# Autodesk Inventor assembly: Gearbox - 54 to 1
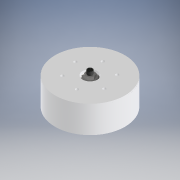
[picture p0: Inventor's stored thumbnail of the model, 180x180]
Saved by Autodesk Inventor 2017 SP1 (Build 210196100, 196)
## iProperties
Created: 2017-09-22
Part Number: Gearbox - 54 to 1
Document SubType Name: Assembly
Designer: Zach
Author: Zach
## Documents named in this file (10)
- C:\Users\Zach\Documents\GitHub\tr1\lib\Gearbox 128;1\Gearbox 128;1.iam
- C:\Users\Zach\Documents\GitHub\tr1\lib\Gearbox 128;1\Base.ipt
- C:\Users\Zach\Documents\GitHub\tr1\lib\22x8x8mm Bearing.ipt
- C:\Users\Zach\Documents\GitHub\tr1\lib\Gearbox 128;1\3mm Brass Rod.ipt
- C:\Users\Zach\Documents\Inventor\Content Center Files\R2017\en-US\ISO 4018\ISO 4018 - M8 x 50.ipt
- C:\Users\Zach\Documents\GitHub\tr1\lib\CNS 3129 - M 8 x 1.25.ipt
- C:\Users\Zach\Documents\GitHub\tr1\lib\Gearbox 128;1\Washer.ipt
- C:\Users\Zach\Documents\GitHub\tr1\lib\Gearbox 128;1\GearSet 1.iam
- C:\Users\Zach\Documents\GitHub\tr1\lib\Gearbox 128;1\Cover.ipt
- C:\Users\Zach\Documents\GitHub\tr1\lib\Gearbox 128;1\Design Accelerator\Spur Gear11.ipt
## Components (34 placed, 9 different names)
1. Base:1 — Mate:1, Flush:1, Mate:4, Flush:2, Mate:5, Flush:3, Mate:6, Flush:4, Mate:7, Flush:5, Mate:8, Flush:6, Mate:9, Flush:7
2. Cover — Mate:155, Flush:14, Mate:157, Rotation:11
3. 22x8x8mm Bearing:1 — Mate:1, Flush:1, Mate:2, Mate:63, Mate:143
4. ISO 4018 M8 x 50:1 — Mate:2, Mate:63, Mate:105, Mate:142, Rotation:7, Mate:155, Mate:156
5. 3mm Brass Rod:1 — Mate:4, Flush:2, Mate:112, Mate:148
6. 3mm Brass Rod:2 — Mate:9, Flush:7, Mate:149
7. 3mm Brass Rod:3 — Mate:8, Flush:6, Mate:138, Mate:140, Mate:144
8. 3mm Brass Rod:4 — Mate:7, Flush:5, Mate:128, Mate:145
9. 3mm Brass Rod:5 — Mate:6, Flush:4, Mate:120, Mate:146
10. 3mm Brass Rod:6 — Mate:5, Flush:3, Mate:114, Mate:147
11. CNS 3129 M 8:1 — Mate:105, Mate:158
12. 22x8x8mm Bearing:2 — Flush:14, Mate:156, Mate:158
13. Washer:1 — Mate:112, Mate:154
14. Washer:2 — Mate:116, Mate:117, Mate:153
15. Washer:3 — Mate:114, Mate:116, Mate:117
16. Washer:4 — Mate:120
17. Washer:5 — Mate:122, Mate:123
18. Washer:6 — Mate:122, Mate:123, Mate:152
19. Washer:7 — Mate:130, Mate:131
20. Washer:8
21. Washer:9 — Mate:128
22. Washer:10 — Mate:130, Mate:131, Mate:151
23. Washer:11
24. Washer:12
25. Washer:13 — Mate:138, Mate:141
26. Washer:14
27. Washer:15 — Mate:140, Mate:141, Mate:150
28. GearSet 1:1 [sub-assembly] — Mate:144, Flush:8, Flush:9, Mate:150, Rotation:1, Rotation:2
29. Spur Gear1:1 — Mate:142, Mate:143, Flush:8, Rotation:1, Rotation:7
30. GearSet 1:2 [sub-assembly] — Mate:145, Flush:9, Flush:10, Mate:151, Rotation:2, Rotation:9
31. GearSet 1:3 [sub-assembly] — Mate:146, Flush:10, Flush:11, Mate:152, Rotation:4, Rotation:9
32. GearSet 1:4 [sub-assembly] — Mate:149, Flush:13, Mate:157, Rotation:10, Rotation:11
33. GearSet 1:5 [sub-assembly] — Mate:148, Flush:12, Flush:13, Mate:154, Rotation:5, Rotation:10
34. GearSet 1:6 [sub-assembly] — Mate:147, Flush:11, Flush:12, Mate:153, Rotation:4, Rotation:5
## Relationships (74: Mate 52, Flush 14, RelateRotation 8)
- Mate:1: Base:1 ↔ 22x8x8mm Bearing:1
- Flush:1: Base:1 ↔ 22x8x8mm Bearing:1
- Mate:2: 22x8x8mm Bearing:1 ↔ ISO 4018 M8 x 50:1
- Mate:4: Base:1 ↔ 3mm Brass Rod:1
- Flush:2: Base:1 ↔ 3mm Brass Rod:1
- Mate:5: Base:1 ↔ 3mm Brass Rod:6
- Flush:3: Base:1 ↔ 3mm Brass Rod:6
- Mate:6: Base:1 ↔ 3mm Brass Rod:5
- Flush:4: Base:1 ↔ 3mm Brass Rod:5
- Mate:7: Base:1 ↔ 3mm Brass Rod:4
- Flush:5: Base:1 ↔ 3mm Brass Rod:4
- Mate:8: Base:1 ↔ 3mm Brass Rod:3
- Flush:6: Base:1 ↔ 3mm Brass Rod:3
- Mate:9: Base:1 ↔ 3mm Brass Rod:2
- Flush:7: Base:1 ↔ 3mm Brass Rod:2
- Mate:63: 22x8x8mm Bearing:1 ↔ ISO 4018 M8 x 50:1
- Mate:105: ISO 4018 M8 x 50:1 ↔ CNS 3129 M 8:1
- Mate:112: 3mm Brass Rod:1 ↔ Washer:1
- Mate:114: 3mm Brass Rod:6 ↔ Washer:3
- Mate:116: Washer:2 ↔ Washer:3
- Mate:117: Washer:2 ↔ Washer:3
- [Mate]: Washer:4 ↔ Washer:5
- [Mate]: Washer:4 ↔ Washer:5
- Mate:120: 3mm Brass Rod:5 ↔ Washer:4
- Mate:122: Washer:5 ↔ Washer:6
- Mate:123: Washer:5 ↔ Washer:6
- [Mate]: Washer:7 ↔ Washer:8
- [Mate]: Washer:7 ↔ Washer:8
- [Mate]: Washer:8 ↔ Washer:9
- [Mate]: Washer:8 ↔ Washer:9
- Mate:128: 3mm Brass Rod:4 ↔ Washer:9
- Mate:130: Washer:7 ↔ Washer:10
- Mate:131: Washer:7 ↔ Washer:10
- [Mate]: Washer:11 ↔ Washer:12
- [Mate]: Washer:11 ↔ Washer:12
- [Mate]: Washer:12 ↔ Washer:13
- [Mate]: Washer:12 ↔ Washer:13
- [Mate]: Washer:11 ↔ Washer:14
- [Mate]: Washer:11 ↔ Washer:14
- Mate:138: 3mm Brass Rod:3 ↔ Washer:13
- Mate:140: 3mm Brass Rod:3 ↔ Washer:15
- Mate:141: Washer:13 ↔ Washer:15
- Mate:142: ISO 4018 M8 x 50:1 ↔ Spur Gear1:1
- Mate:143: 22x8x8mm Bearing:1 ↔ Spur Gear1:1
- Mate:144: 3mm Brass Rod:3 ↔ GearSet 1:1
- Flush:8: GearSet 1:1 ↔ Spur Gear1:1
- Mate:145: 3mm Brass Rod:4 ↔ GearSet 1:2
- Flush:9: GearSet 1:1 ↔ GearSet 1:2
- Mate:146: 3mm Brass Rod:5 ↔ GearSet 1:3
- Flush:10: GearSet 1:2 ↔ GearSet 1:3
- Mate:147: 3mm Brass Rod:6 ↔ GearSet 1:6
- Flush:11: GearSet 1:3 ↔ GearSet 1:6
- Mate:148: 3mm Brass Rod:1 ↔ GearSet 1:5
- Flush:12: GearSet 1:5 ↔ GearSet 1:6
- Mate:149: 3mm Brass Rod:2 ↔ GearSet 1:4
- Flush:13: GearSet 1:4 ↔ GearSet 1:5
- Mate:150: Washer:15 ↔ GearSet 1:1
- Mate:151: Washer:10 ↔ GearSet 1:2
- Mate:152: Washer:6 ↔ GearSet 1:3
- Mate:153: Washer:2 ↔ GearSet 1:6
- Mate:154: Washer:1 ↔ GearSet 1:5
- Rotation:1 [RelateRotation] (0.5 ul): GearSet 1:1 ↔ Spur Gear1:1
- Rotation:2 [RelateRotation] (0.5 ul): GearSet 1:1 ↔ GearSet 1:2
- Rotation:4 [RelateRotation] (0.5 ul): GearSet 1:3 ↔ GearSet 1:6
- Rotation:5 [RelateRotation] (0.5 ul): GearSet 1:5 ↔ GearSet 1:6
- Rotation:7 [RelateRotation] (1 ul): ISO 4018 M8 x 50:1 ↔ Spur Gear1:1
- Mate:155: Cover ↔ ISO 4018 M8 x 50:1
- Flush:14: Cover ↔ 22x8x8mm Bearing:2
- Mate:156: ISO 4018 M8 x 50:1 ↔ 22x8x8mm Bearing:2
- Mate:157: Cover ↔ GearSet 1:4
- Rotation:9 [RelateRotation] (0.5 ul): GearSet 1:2 ↔ GearSet 1:3
- Rotation:10 [RelateRotation] (0.5 ul): GearSet 1:4 ↔ GearSet 1:5
- Rotation:11 [RelateRotation] (0.5 ul): Cover ↔ GearSet 1:4
- Mate:158: CNS 3129 M 8:1 ↔ 22x8x8mm Bearing:2
## Named parameters: d143_d141 = 0 mm, d144_d142 = 0 mm, d149_d143_d141 = 0 mm, d150_d144_d142 = 0 mm, d151_d147 = 0 mm, d152_d148 = 0 mm, d157_d149_d143_d141 = 0 mm, d158_d150_d144_d142 = 0 mm, d159_d151_d147 = 0 mm, d160_d152_d148 = 0 mm, d161_d155 = 0 mm, d162_d156 = 0 mm
